# Autodesk Inventor assembly: base
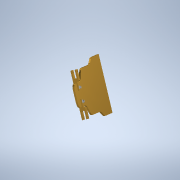
[picture p0: Inventor's stored thumbnail of the model, 180x180]
Saved by Autodesk Inventor 2020 (Build 240168000, 168)
## iProperties
Created: 2020-03-15
Part Number: base
Document SubType Name: Assembly
Designer: 0x6f736f646f
Author: 0x6f736f646f
## Documents named in this file (5)
- C:\Users\0x6f736f646f\Documents\EurekaAutonomousCar\Src\Prototyping\Mechanical\chassis_version_2\base.iam
- C:\Users\0x6f736f646f\Documents\EurekaAutonomousCar\Src\Prototyping\Mechanical\chassis_version_2\1.ipt
- C:\Users\0x6f736f646f\Documents\EurekaAutonomousCar\Src\Prototyping\Mechanical\chassis_version_2\2.ipt
- C:\Users\0x6f736f646f\Documents\EurekaAutonomousCar\Src\Prototyping\Mechanical\chassis_ver1\Content Center\en-US\ANSI B 18.6.7 M IFI 513(2)\ANSI B 18.6.7 M _ IFI 513 - M3x0.5 x 10(1).ipt
- C:\Users\0x6f736f646f\Documents\EurekaAutonomousCar\Src\Prototyping\Mechanical\chassis_ver1\Content Center\en-US\ANSI B 18.2.4.1 M(1)\ANSI B 18.2.4.1 M - M3 x 0.5Style 1.ipt
## Components (8 placed, 4 different names)
1. 1:1 — Mate:1, Mate:2, Mate:3, Mate:4, Mate:5, Mate:6, Mate:8
2. 2:1 — Mate:1, Mate:3, Mate:5, Mate:7, Mate:9, Mate:15
3. 2:2 — Mate:2, Mate:4, Mate:6, Mate:10, Mate:13
4. Hex Flange Head Machine Screw - Metric M3x0.5 x 10:1 — Mate:8, Mate:10, Mate:11
5. Hex Flange Head Machine Screw - Metric M3x0.5 x 10:2 — Mate:7, Mate:9, Mate:12, Mate:14
6. Hex Nut Metric M3 x 0.5:1 — Mate:11, Mate:13
7. Hex Nut Metric M3 x 0.5:2 — Mate:12
8. Hex Nut Metric M3 x 0.5:3 — Mate:14, Mate:15
## Relationships (15: Mate 15)
- Mate:1: 1:1 ↔ 2:1
- Mate:2: 1:1 ↔ 2:2
- Mate:3: 1:1 ↔ 2:1
- Mate:4: 1:1 ↔ 2:2
- Mate:5: 1:1 ↔ 2:1
- Mate:6: 1:1 ↔ 2:2
- Mate:7: 2:1 ↔ Hex Flange Head Machine Screw - Metric M3x0.5 x 10:2
- Mate:8: 1:1 ↔ Hex Flange Head Machine Screw - Metric M3x0.5 x 10:1
- Mate:9: 2:1 ↔ Hex Flange Head Machine Screw - Metric M3x0.5 x 10:2
- Mate:10: 2:2 ↔ Hex Flange Head Machine Screw - Metric M3x0.5 x 10:1
- Mate:11: Hex Flange Head Machine Screw - Metric M3x0.5 x 10:1 ↔ Hex Nut Metric M3 x 0.5:1
- Mate:12: Hex Flange Head Machine Screw - Metric M3x0.5 x 10:2 ↔ Hex Nut Metric M3 x 0.5:2
- Mate:13: 2:2 ↔ Hex Nut Metric M3 x 0.5:1
- Mate:14: Hex Flange Head Machine Screw - Metric M3x0.5 x 10:2 ↔ Hex Nut Metric M3 x 0.5:3
- Mate:15: 2:1 ↔ Hex Nut Metric M3 x 0.5:3
